# Autodesk Inventor assembly: PS20028
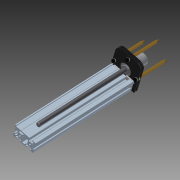
[picture p0: Inventor's stored thumbnail of the model, 180x180]
Saved by Autodesk Inventor 2014 (Build 180170000, 170)
## iProperties
Created: 2013-11-25
Part Number: PS20028
Document SubType Name: Assembly
Designer: Edward
Description: Z-Axis Rail Assembly
Author: Edward
Title: Z-Axis Rail Assembly
Subject: Shapeoko 2
## Documents named in this file (15)
- C:\Users\Edward\Documents\GitHub\Shapeoko_2\Autodesk_Inventor_Project\PS20028.iam
- C:\Users\Edward\Documents\GitHub\Shapeoko_2\Autodesk_Inventor_Project\25142-07.ipt
- C:\Users\Edward\Documents\GitHub\Shapeoko_2\Autodesk_Inventor_Project\25772-02.ipt
- C:\Users\Edward\Documents\GitHub\Shapeoko_2\Autodesk_Inventor_Project\30288-01.ipt
- C:\Users\Edward\Documents\GitHub\Shapeoko_2\Autodesk_Inventor_Project\30169-01.ipt
- C:\Users\Edward\Documents\GitHub\Shapeoko_2\Autodesk_Inventor_Project\30289-01.ipt
- C:\Users\Edward\Documents\GitHub\Shapeoko_2\Autodesk_Inventor_Project\PS20011.ipt
- C:\Users\Edward\Documents\GitHub\Shapeoko_2\Autodesk_Inventor_Project\25287-02.ipt
- C:\Users\Edward\Documents\GitHub\Shapeoko_2\Autodesk_Inventor_Project\PS20014.ipt
- C:\Users\Edward\Documents\GitHub\Shapeoko_2\Autodesk_Inventor_Project\PS20016.ipt
- C:\Users\Edward\Documents\GitHub\Shapeoko_2\Autodesk_Inventor_Project\PS20004.ipt
- C:\Users\Edward\Documents\GitHub\Shapeoko_2\Autodesk_Inventor_Project\PS20015.ipt
- C:\Users\Edward\Documents\GitHub\Shapeoko_2\Autodesk_Inventor_Project\25285-10.ipt
- C:\Users\Edward\Documents\GitHub\Shapeoko_2\Autodesk_Inventor_Project\25287-03.ipt
- C:\Users\Edward\Documents\GitHub\Shapeoko_2\Autodesk_Inventor_Project\PS20007.ipt
## Components (32 placed, 14 different names)
1. 25142-07:1 — Insert:12, Insert:13
2. PS20014:2 — Insert:30
3. 25287-02:3 — Insert:24, Insert:29
4. PS20004:3
5. 30289-01:3 — Insert:12, Insert:13, Mate:1, Flush:1, Insert:24, Mate:2, Flush:2
6. 30288-01:4 — Mate:1, Flush:1, Insert:14, Insert:16, Insert:18, Flush:2, Insert:37, Insert:38, Insert:39
7. PS20016:6 — Insert:26, Insert:27
8. 30169-01:3 — Insert:23, Mate:4, Flush:3, Insert:40, Insert:41
9. 30288-01:5 — Insert:20, Insert:21, Insert:22, Insert:23, Mate:3, Insert:30, Insert:31, Insert:32
10. 25772-02:3 — Insert:33
11. PS20011:3 — Mate:4, Flush:3, Insert:33
12. PS20015:1 — Insert:14, Insert:15
13. PS20015:2 — Insert:15, Insert:22
14. PS20015:3 — Insert:16, Insert:17
15. PS20015:4 — Insert:17, Insert:20
16. PS20015:5 — Insert:18, Insert:19
17. PS20015:6 — Insert:19, Insert:21
18. 25287-02:4 — Insert:26, Mate:3
19. PS20004:4
20. PS20016:7 — Insert:27, Mate:2
21. PS20016:8 — Insert:29
22. PS20016:9
23. PS20014:3 — Insert:31
24. PS20014:4 — Insert:32
25. 25285-10:1 — Insert:34
26. 25287-03:1 — Insert:34, Insert:37
27. 25285-10:2
28. 25287-03:2 — Insert:39
29. 25285-10:3
30. 25287-03:3 — Insert:38
31. PS20007:1 — Insert:40
32. PS20007:2 — Insert:41
## Relationships (38: Insert 31, Mate 4, Flush 3)
- [Insert]: 25287-02:3 ↔ PS20004:3
- Insert:12: 25142-07:1 ↔ 30289-01:3
- Insert:13: 25142-07:1 ↔ 30289-01:3
- Mate:1: 30289-01:3 ↔ 30288-01:4
- Flush:1 (-5 mm): 30289-01:3 ↔ 30288-01:4
- Insert:14: 30288-01:4 ↔ PS20015:1
- Insert:15: PS20015:1 ↔ PS20015:2
- Insert:16: 30288-01:4 ↔ PS20015:3
- Insert:17: PS20015:3 ↔ PS20015:4
- Insert:18: 30288-01:4 ↔ PS20015:5
- Insert:19: PS20015:5 ↔ PS20015:6
- Insert:20: 30288-01:5 ↔ PS20015:4
- Insert:21: 30288-01:5 ↔ PS20015:6
- Insert:22: 30288-01:5 ↔ PS20015:2
- Insert:23: 30169-01:3 ↔ 30288-01:5
- Insert:24 (7.3137 mm): 25287-02:3 ↔ 30289-01:3
- [Insert]: 25287-02:4 ↔ PS20004:4
- Insert:26 (3.4163 mm): PS20016:6 ↔ 25287-02:4
- Insert:27: PS20016:6 ↔ PS20016:7
- [Insert]: PS20016:8 ↔ PS20016:9
- Insert:29 (3.4163 mm): 25287-02:3 ↔ PS20016:8
- Mate:2: 30289-01:3 ↔ PS20016:7
- Mate:3: 30288-01:5 ↔ 25287-02:4
- Flush:2: 30289-01:3 ↔ 30288-01:4
- Insert:30: PS20014:2 ↔ 30288-01:5
- Insert:31: 30288-01:5 ↔ PS20014:3
- Insert:32: 30288-01:5 ↔ PS20014:4
- Mate:4: 30169-01:3 ↔ PS20011:3
- Flush:3 (-10 mm): 30169-01:3 ↔ PS20011:3
- Insert:33 (1 mm): 25772-02:3 ↔ PS20011:3
- Insert:34: 25285-10:1 ↔ 25287-03:1
- [Insert]: 25285-10:2 ↔ 25287-03:2
- [Insert]: 25285-10:3 ↔ 25287-03:3
- Insert:37: 30288-01:4 ↔ 25287-03:1
- Insert:38: 30288-01:4 ↔ 25287-03:3
- Insert:39: 30288-01:4 ↔ 25287-03:2
- Insert:40: 30169-01:3 ↔ PS20007:1
- Insert:41: 30169-01:3 ↔ PS20007:2
## Named parameters: d18_d15_d212_d101_d55_d51 = 0 mm, d35_d18_d15_d212_d101_d55_d51 = 0 mm, d38_d37 = 0 mm, d50_d49 = 0 mm, d51_d49 = 0 mm
